# Autodesk Inventor assembly: NMRV30_motor
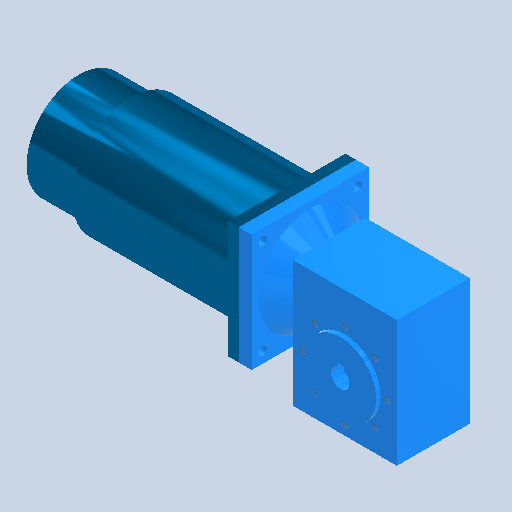
[picture p0: Inventor's stored thumbnail of the model, 512x512]
Saved by Autodesk Inventor 2025.3 (Build 293356030, 356C)
## iProperties
Created: 2025-08-25
Part Number: NMRV30_motor
Document SubType Name: Assembly
Designer: MSI
Mass: 6000 g
Surface Area: 1241.78 cm^2
Volume: 1593.93 cm^3
Author: MSI
## Documents named in this file (3)
- C:\Users\MSI\Desktop\Project\3. 로봇팔\Robot Arm Model\Robot_Arm_6_v1\NMRV30_motor.iam
- C:\Users\MSI\Desktop\Project\3. 로봇팔\Robot Arm Model\Robot_Arm_6_v1\motor.ipt
- C:\Users\MSI\Desktop\Project\3. 로봇팔\Robot Arm Model\Robot_Arm_6_v1\motor_gear_head.ipt
## Components (2 placed, 2 different names)
1. motor:1 — 강체:1
2. motor_gear_head:1 — 강체:1
## Relationships (1: WeldJoint 1)
- 강체:1 [WeldJoint]: motor:1 ↔ motor_gear_head:1
